# Autodesk Inventor assembly: AM14U3 Square Frame Half
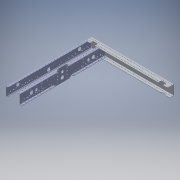
[picture p0: Inventor's stored thumbnail of the model, 180x180]
Saved by Autodesk Inventor 2016 (Build 200138000, 138)
## iProperties
Created: 2016-01-27
Part Number: AM14U3 Square Frame Half
Document SubType Name: Assembly
Designer: PrashantBIA
Author: PrashantBIA
Revision Number: ANY
## Documents named in this file (4)
- C:\Users\Andrew\Documents\GitHub\2016RobotCADFiles\Drive Train\AM14U3 Square Frame Half.iam
- C:\Users\Andrew\Documents\GitHub\2016RobotCADFiles\Drive Train\AM14U3 End Sheet Square.ipt
- C:\Users\Andrew\Documents\GitHub\2016RobotCADFiles\Drive Train\AM14U3 Inside Sheet Square.ipt
- C:\Users\Andrew\Documents\GitHub\2016RobotCADFiles\Drive Train\AM14U3 Outside Sheet Square.ipt
## Components (3 placed, 3 different names)
1. AM14U3 End Sheet Square_125 — Mate:3, Mate:4, Mate:5
2. AM14U3 Inside Sheet Square_126 — Mate:1, Flush:1, Flush:2
3. AM14U3 Outside Sheet Square_127 — Mate:1, Flush:1, Flush:2, Mate:3, Mate:4, Mate:5
## Relationships (6: Mate 4, Flush 2)
- Mate:1 (111.125 mm): AM14U3 Inside Sheet Square_126 ↔ AM14U3 Outside Sheet Square_127
- Flush:1: AM14U3 Inside Sheet Square_126 ↔ AM14U3 Outside Sheet Square_127
- Flush:2: AM14U3 Inside Sheet Square_126 ↔ AM14U3 Outside Sheet Square_127
- Mate:3: AM14U3 End Sheet Square_125 ↔ AM14U3 Outside Sheet Square_127
- Mate:4: AM14U3 End Sheet Square_125 ↔ AM14U3 Outside Sheet Square_127
- Mate:5: AM14U3 End Sheet Square_125 ↔ AM14U3 Outside Sheet Square_127
